# Autodesk Inventor assembly: ASY ANP 1424 FDS way 4
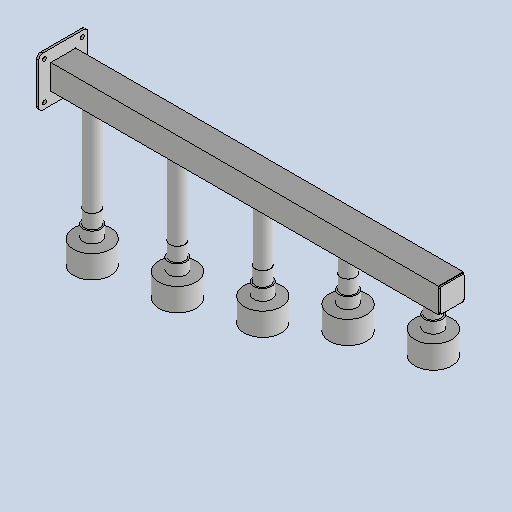
[picture p0: Inventor's stored thumbnail of the model, 512x512]
Saved by Autodesk Inventor 2025.3 (Build 293356030, 356C)
## iProperties
Created: 2025-07-02
Part Number: ASY ANP 1424 FDS way 4
Document SubType Name: Assembly
Designer: admin
Author: user
## Documents named in this file (10)
- C:\Users\admin\Yandex.Disk\home pc\Inventor\ANP--Antipayuta\FDS 1400\ASY ANP 1424 FDS way 4.iam
- C:\Users\admin\Yandex.Disk\home pc\Inventor\ANP--Antipayuta\FDS 1400\ANP 1434 FDS WAY tube4.ipt
- C:\Users\admin\Yandex.Disk\home pc\Inventor\ANP--Antipayuta\FDS 1400\ANP 1425 FDS Way FLANGE.ipt
- C:\Users\admin\Yandex.Disk\home pc\Inventor\ANP--Antipayuta\FDS 1400\ANP 1426 FDS way cup.ipt
- C:\Users\admin\Yandex.Disk\home pc\Inventor\ANP--Antipayuta\FDS 1400\ANP dummy filter element.ipt
- C:\Users\admin\Yandex.Disk\home pc\Inventor\ANP--Antipayuta\FDS 1400\ANP dummy pipe nippel.ipt
- C:\Users\admin\Yandex.Disk\home pc\Inventor\ANP--Antipayuta\FDS 1400\ANP 1447 FDS thread  tube7.ipt
- C:\Users\admin\Yandex.Disk\home pc\Inventor\ANP--Antipayuta\FDS 1400\ANP 1448 FDS thread  tube8.ipt
- C:\Users\admin\Yandex.Disk\home pc\Inventor\ANP--Antipayuta\FDS 1400\ANP 1449 FDS thread  tube9.ipt
- C:\Users\admin\Yandex.Disk\home pc\Inventor\ANP--Antipayuta\FDS 1400\ANP 1451 FDS thread  tube10.ipt
## Components (17 placed, 9 different names)
1. ANP 1434 FDS WAY tube4.ipt:1 — Rigid:34, Rigid:35, Rigid:36, Rigid:52, Rigid:53, Rigid:54, Rigid:55
2. ANP 1425 FDS Way FLANGE.ipt:1 — Rigid:34
3. ANP 1426 FDS way cup.ipt:1 — Rigid:35
4. ANP dummy filter element.ipt:1 — Rigid:1
5. ANP dummy pipe nippel.ipt:1 — Rigid:1, Rigid:44
6. ANP dummy filter element.ipt:2 — Rigid:6
7. ANP dummy pipe nippel.ipt:2 — Rigid:6, Rigid:46
8. ANP dummy filter element.ipt:3 — Rigid:11
9. ANP dummy pipe nippel.ipt:3 — Rigid:11, Rigid:47
10. ANP dummy filter element.ipt:4 — Rigid:14
11. ANP dummy pipe nippel.ipt:4 — Rigid:14, Rigid:45
12. ANP dummy filter element.ipt:5 — Rigid:33
13. ANP dummy pipe nippel.ipt:5 — Rigid:36, Rigid:33
14. ANP 1447 FDS thread  tube7.ipt:1 — Rigid:52, Rigid:47
15. ANP 1448 FDS thread  tube8.ipt:1 — Rigid:53, Rigid:46
16. ANP 1449 FDS thread  tube9.ipt:1 — Rigid:54, Rigid:45
17. ANP 1451 FDS thread  tube10.ipt:1 — Rigid:55, Rigid:44
## Relationships (16: WeldJoint 16)
- Rigid:1 [WeldJoint]: ANP dummy filter element.ipt:1 ↔ ANP dummy pipe nippel.ipt:1
- Rigid:6 [WeldJoint]: ANP dummy filter element.ipt:2 ↔ ANP dummy pipe nippel.ipt:2
- Rigid:34 [WeldJoint] (2 mm): ANP 1434 FDS WAY tube4.ipt:1 ↔ ANP 1425 FDS Way FLANGE.ipt:1
- Rigid:35 [WeldJoint]: ANP 1434 FDS WAY tube4.ipt:1 ↔ ANP 1426 FDS way cup.ipt:1
- Rigid:11 [WeldJoint]: ANP dummy filter element.ipt:3 ↔ ANP dummy pipe nippel.ipt:3
- Rigid:14 [WeldJoint]: ANP dummy filter element.ipt:4 ↔ ANP dummy pipe nippel.ipt:4
- Rigid:36 [WeldJoint]: ANP 1434 FDS WAY tube4.ipt:1 ↔ ANP dummy pipe nippel.ipt:5
- Rigid:33 [WeldJoint]: ANP dummy filter element.ipt:5 ↔ ANP dummy pipe nippel.ipt:5
- Rigid:52 [WeldJoint]: ANP 1434 FDS WAY tube4.ipt:1 ↔ ANP 1447 FDS thread  tube7.ipt:1
- Rigid:47 [WeldJoint]: ANP dummy pipe nippel.ipt:3 ↔ ANP 1447 FDS thread  tube7.ipt:1
- Rigid:53 [WeldJoint]: ANP 1434 FDS WAY tube4.ipt:1 ↔ ANP 1448 FDS thread  tube8.ipt:1
- Rigid:46 [WeldJoint]: ANP dummy pipe nippel.ipt:2 ↔ ANP 1448 FDS thread  tube8.ipt:1
- Rigid:54 [WeldJoint]: ANP 1434 FDS WAY tube4.ipt:1 ↔ ANP 1449 FDS thread  tube9.ipt:1
- Rigid:45 [WeldJoint]: ANP dummy pipe nippel.ipt:4 ↔ ANP 1449 FDS thread  tube9.ipt:1
- Rigid:55 [WeldJoint]: ANP 1434 FDS WAY tube4.ipt:1 ↔ ANP 1451 FDS thread  tube10.ipt:1
- Rigid:44 [WeldJoint]: ANP dummy pipe nippel.ipt:1 ↔ ANP 1451 FDS thread  tube10.ipt:1
